# Autodesk Inventor assembly: switch
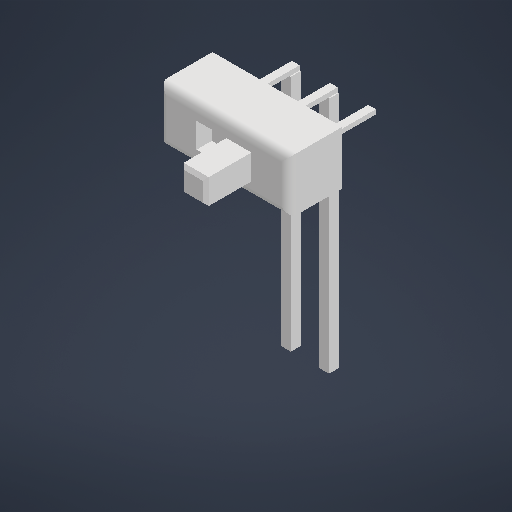
[picture p0: Inventor's stored thumbnail of the model, 512x512]
Saved by Autodesk Inventor 2025.2 (Build 292293000, 293)
## iProperties
Created: 2025-12-13
Part Number: switch
Document SubType Name: Assembly
Designer: sam
Author: sam
## Documents named in this file (3)
- G:\projects\primary\regulated-irrigation-system\model\asm\pcb\switch\switch.iam
- G:\projects\primary\regulated-irrigation-system\model\asm\pcb\switch\switch.ipt
- G:\projects\primary\regulated-irrigation-system\model\asm\pcb\switch\switch-wire.ipt
## Components (3 placed, 2 different names)
1. switch:1 — Mate:1, Flush:1, Flush:2, Mate:2, Flush:3, Flush:4
2. switch-wire:1 — Mate:1, Flush:1, Flush:2
3. switch-wire:2 — Mate:2, Flush:3, Flush:4
## Relationships (6: Flush 4, Mate 2)
- Mate:1: switch:1 ↔ switch-wire:1
- Flush:1: switch:1 ↔ switch-wire:1
- Flush:2 (-0.07 mm): switch:1 ↔ switch-wire:1
- Mate:2: switch:1 ↔ switch-wire:2
- Flush:3: switch:1 ↔ switch-wire:2
- Flush:4 (-0.07 mm): switch:1 ↔ switch-wire:2
